# Autodesk Inventor assembly: Mellie Side Cart
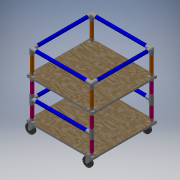
[picture p0: Inventor's stored thumbnail of the model, 180x180]
Saved by Autodesk Inventor 2018.2 (Build 222227000, 227)
## iProperties
Created: 2018-03-20
Part Number: Mellie Side Cart
Document SubType Name: Assembly
Designer: owner
Author: owner
## Documents named in this file (10)
- Z:\The Pickle - 4 - Copy\Final Carts\Mellie Cart\Mellie Side Cart.iam
- Z:\The Pickle - 4 - Copy\Final Carts\Mellie Cart\Mellie Side Plywood Base.ipt
- Z:\The Pickle - 4 - Copy\Final Carts\Mellie Cart\Mellie Pipe 1 (Main and Side).ipt
- Z:\The Pickle - 4 - Copy\Final Carts\Mellie Cart\Mellie Side Pipe 6.ipt
- Z:\The Pickle - 4 - Copy\Final Carts\Stuff Used By All Carts\PVC Fittings (Formufit)\Wood Mount 1 Inch.ipt
- Z:\The Pickle - 4 - Copy\Final Carts\Stuff Used By All Carts\PVC Fittings (Formufit)\3-way 90 1 Inch.ipt
- Z:\The Pickle - 4 - Copy\Final Carts\Stuff Used By All Carts\PVC Fittings (Formufit)\4-way Tee 1 Inch.ipt
- Z:\The Pickle - 4 - Copy\Final Carts\Stuff Used By All Carts\PVC Fittings (Formufit)\Tee 1 Inch.ipt
- Z:\The Pickle - 4 - Copy\Final Carts\Stuff Used By All Carts\WHEELS.ipt
- Z:\The Pickle - 4 - Copy\Final Carts\Mellie Cart\Mellie Side Pipe 5.ipt
## Components (45 placed, 9 different names)
1. Mellie Side Plywood Base:1 — Mate:1, Tangent:1, Tangent:2, Tangent:3, Flush:1, Flush:2, Flush:10, Flush:11, Flush:12, Flush:13, Mate:4
2. Mellie Side Plywood Base:2 — Mate:2, Flush:1, Flush:2, Mate:3, Tangent:4, Tangent:5, Tangent:6
3. Mellie Pipe 1 (Main and Side):1 — Insert:32, Insert:33
4. Mellie Pipe 1 (Main and Side):2 — Insert:28, Insert:29
5. Mellie Pipe 1 (Main and Side):3 — Insert:18, Insert:19
6. Mellie Pipe 1 (Main and Side):4 — Insert:14, Insert:15
7. Mellie Pipe 1 (Main and Side):5 — Insert:16, Insert:17
8. Mellie Pipe 1 (Main and Side):6 — Insert:30, Insert:31
9. Mellie Pipe 1 (Main and Side):7 — Insert:34
10. Mellie Side Pipe 6:1 — Insert:7, Insert:21
11. Mellie Side Pipe 6:2 — Insert:10, Insert:24
12. Mellie Side Pipe 6:3 — Insert:11, Insert:25
13. Mellie Side Pipe 6:4 — Insert:12, Insert:26
14. Mellie Side Pipe 6:5 — Insert:9, Insert:23
15. Mellie Side Pipe 6:6 — Insert:8, Insert:22
16. Mellie Side Pipe 6:7 — Insert:2, Insert:20
17. Mellie Side Pipe 6:8 — Insert:1, Insert:13
18. Mellie Side Pipe 5:1 — Insert:4, Insert:35
19. Mellie Side Pipe 5:2 — Insert:5, Insert:36
20. Mellie Side Pipe 5:3 — Insert:6, Insert:37
21. Mellie Side Pipe 5:4 — Insert:3, Insert:27
22. Wood Mount 1 Inch:1 — Mate:1, Tangent:1, Tangent:2, Tangent:3, Insert:1
23. Wood Mount 1 Inch:2 — Insert:2
24. Wood Mount 1 Inch:3 — Insert:3, Mate:3, Tangent:4, Tangent:5, Tangent:6
25. Wood Mount 1 Inch:4 — Insert:4
26. Wood Mount 1 Inch:5 — Insert:5
27. Wood Mount 1 Inch:6 — Insert:6
28. Wood Mount 1 Inch:7 — Insert:7
29. Wood Mount 1 Inch:8 — Insert:8
30. Wood Mount 1 Inch:9 — Insert:9
31. Wood Mount 1 Inch:10 — Insert:10
32. Wood Mount 1 Inch:11 — Insert:11, Mate:2
33. Wood Mount 1 Inch:12 — Insert:12
34. 3-way 90 1 Inch:1 — Insert:31, Insert:32, Insert:36
35. 3-way 90 1 Inch:2 — Insert:33, Insert:34, Insert:37
36. 3-way 90 1 Inch:3 — Insert:27, Insert:28
37. 3-way 90 1 Inch:4 — Insert:29, Insert:30, Insert:35
38. 4-way Tee 1 Inch:1 — Insert:17, Insert:18, Insert:21, Insert:24
39. 4-way Tee 1 Inch:2 — Insert:15, Insert:16, Insert:20, Insert:26
40. Tee 1 Inch:2 — Insert:19, Insert:22, Insert:23
41. Tee 1 Inch:3 — Insert:13, Insert:14, Insert:25
42. WHEELS:1 — Flush:5, Flush:8, Flush:9
43. WHEELS:2 — Flush:4, Flush:5, Flush:7, Flush:9, Flush:12, Flush:13, Mate:4
44. WHEELS:3 — Flush:3, Flush:4, Flush:6, Flush:7
45. WHEELS:4 — Flush:3, Flush:6, Flush:8, Flush:10, Flush:11
## Relationships (60: Insert 37, Flush 13, Tangent 6, Mate 4)
- Mate:1: Mellie Side Plywood Base:1 ↔ Wood Mount 1 Inch:1
- Tangent:1: Mellie Side Plywood Base:1 ↔ Wood Mount 1 Inch:1
- Tangent:2: Mellie Side Plywood Base:1 ↔ Wood Mount 1 Inch:1
- Tangent:3: Mellie Side Plywood Base:1 ↔ Wood Mount 1 Inch:1
- Insert:1: Mellie Side Pipe 6:8 ↔ Wood Mount 1 Inch:1
- Insert:2: Mellie Side Pipe 6:7 ↔ Wood Mount 1 Inch:2
- Insert:3: Mellie Side Pipe 5:4 ↔ Wood Mount 1 Inch:3
- Insert:4: Mellie Side Pipe 5:1 ↔ Wood Mount 1 Inch:4
- Insert:5: Mellie Side Pipe 5:2 ↔ Wood Mount 1 Inch:5
- Insert:6: Mellie Side Pipe 5:3 ↔ Wood Mount 1 Inch:6
- Insert:7: Mellie Side Pipe 6:1 ↔ Wood Mount 1 Inch:7
- Insert:8: Mellie Side Pipe 6:6 ↔ Wood Mount 1 Inch:8
- Insert:9: Mellie Side Pipe 6:5 ↔ Wood Mount 1 Inch:9
- Insert:10: Mellie Side Pipe 6:2 ↔ Wood Mount 1 Inch:10
- Insert:11: Mellie Side Pipe 6:3 ↔ Wood Mount 1 Inch:11
- Insert:12: Mellie Side Pipe 6:4 ↔ Wood Mount 1 Inch:12
- Insert:13: Mellie Side Pipe 6:8 ↔ Tee 1 Inch:3
- Insert:14: Mellie Pipe 1 (Main and Side):4 ↔ Tee 1 Inch:3
- Insert:15: Mellie Pipe 1 (Main and Side):4 ↔ 4-way Tee 1 Inch:2
- Insert:16: Mellie Pipe 1 (Main and Side):5 ↔ 4-way Tee 1 Inch:2
- Insert:17: Mellie Pipe 1 (Main and Side):5 ↔ 4-way Tee 1 Inch:1
- Insert:18: Mellie Pipe 1 (Main and Side):3 ↔ 4-way Tee 1 Inch:1
- Insert:19: Mellie Pipe 1 (Main and Side):3 ↔ Tee 1 Inch:2
- Insert:20: Mellie Side Pipe 6:7 ↔ 4-way Tee 1 Inch:2
- Insert:21: Mellie Side Pipe 6:1 ↔ 4-way Tee 1 Inch:1
- Insert:22: Mellie Side Pipe 6:6 ↔ Tee 1 Inch:2
- Insert:23: Mellie Side Pipe 6:5 ↔ Tee 1 Inch:2
- Insert:24: Mellie Side Pipe 6:2 ↔ 4-way Tee 1 Inch:1
- Insert:25: Mellie Side Pipe 6:3 ↔ Tee 1 Inch:3
- Insert:26: Mellie Side Pipe 6:4 ↔ 4-way Tee 1 Inch:2
- Mate:2: Mellie Side Plywood Base:2 ↔ Wood Mount 1 Inch:11
- Flush:1: Mellie Side Plywood Base:1 ↔ Mellie Side Plywood Base:2
- Flush:2: Mellie Side Plywood Base:1 ↔ Mellie Side Plywood Base:2
- Mate:3: Mellie Side Plywood Base:2 ↔ Wood Mount 1 Inch:3
- Tangent:4: Mellie Side Plywood Base:2 ↔ Wood Mount 1 Inch:3
- Tangent:5: Mellie Side Plywood Base:2 ↔ Wood Mount 1 Inch:3
- Tangent:6: Mellie Side Plywood Base:2 ↔ Wood Mount 1 Inch:3
- Insert:27: Mellie Side Pipe 5:4 ↔ 3-way 90 1 Inch:3
- Insert:28: Mellie Pipe 1 (Main and Side):2 ↔ 3-way 90 1 Inch:3
- Insert:29: Mellie Pipe 1 (Main and Side):2 ↔ 3-way 90 1 Inch:4
- Insert:30: Mellie Pipe 1 (Main and Side):6 ↔ 3-way 90 1 Inch:4
- Insert:31: Mellie Pipe 1 (Main and Side):6 ↔ 3-way 90 1 Inch:1
- Insert:32: Mellie Pipe 1 (Main and Side):1 ↔ 3-way 90 1 Inch:1
- Insert:33: Mellie Pipe 1 (Main and Side):1 ↔ 3-way 90 1 Inch:2
- Insert:34: Mellie Pipe 1 (Main and Side):7 ↔ 3-way 90 1 Inch:2
- Insert:35: Mellie Side Pipe 5:1 ↔ 3-way 90 1 Inch:4
- Insert:36: Mellie Side Pipe 5:2 ↔ 3-way 90 1 Inch:1
- Insert:37: Mellie Side Pipe 5:3 ↔ 3-way 90 1 Inch:2
- Flush:3: WHEELS:3 ↔ WHEELS:4
- Flush:4: WHEELS:2 ↔ WHEELS:3
- Flush:5: WHEELS:1 ↔ WHEELS:2
- Flush:6: WHEELS:3 ↔ WHEELS:4
- Flush:7: WHEELS:2 ↔ WHEELS:3
- Flush:8: WHEELS:1 ↔ WHEELS:4
- Flush:9: WHEELS:1 ↔ WHEELS:2
- Flush:10: Mellie Side Plywood Base:1 ↔ WHEELS:4
- Flush:11: Mellie Side Plywood Base:1 ↔ WHEELS:4
- Flush:12: Mellie Side Plywood Base:1 ↔ WHEELS:2
- Flush:13: Mellie Side Plywood Base:1 ↔ WHEELS:2
- Mate:4: Mellie Side Plywood Base:1 ↔ WHEELS:2
